# Autodesk Inventor assembly: REAR RIGHT BUKHEAD
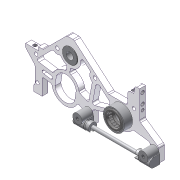
[picture p0: Inventor's stored thumbnail of the model, 180x180]
Saved by Autodesk Inventor 2016 (Build 200138000, 138)
## iProperties
Created: 2015-04-18
Part Number: REAR RIGHT BUKHEAD
Document SubType Name: Assembly
Designer: Station9
Author: Station9
## Documents named in this file (10)
- E:\worldskills Project\Project Archive\AD\AD-6(94.01.29)WSC2011\REAR RIGHT BUKHEAD.iam
- E:\worldskills Project\Project Archive\AD\AD-6(94.01.29)WSC2011\500-171.ipt
- E:\worldskills Project\Project Archive\AD\AD-6(94.01.29)WSC2011\500-172.ipt
- E:\worldskills Project\Project Archive\AD\AD-6(94.01.29)WSC2011\500-168.ipt
- E:\worldskills Project\Project Archive\AD\AD-6(94.01.29)WSC2011\500-160.ipt
- E:\worldskills Project\Project Archive\AD\AD-6(94.01.29)WSC2011\500-125.ipt
- E:\worldskills Project\Project Archive\AD\AD-6(94.01.29)WSC2011\500-169.ipt
- E:\worldskills Project\Project Archive\AD\AD-6(94.01.29)WSC2011\500-136.ipt
- E:\worldskills Project\Project Archive\AD\AD-6(94.01.29)WSC2011\Content Center\en-US\ISO 3245 (I)\ISO 3245 - 21 D - 12 x 16 x 7(1) I.ipt
- E:\worldskills Project\Project Archive\AD\AD-6(94.01.29)WSC2011\Bulkhead_RR.ipt
## Components (11 placed, 9 different names)
1. 500-171:1 — Mate:6, Mate:9, Mate:17, Mate:19
2. 500-172:1 — Mate:5, Mate:7, Mate:15, Mate:16, Mate:18
3. 500-168:1 — Mate:8, Mate:9, Mate:11, Angle:1
4. 500-160:1 — Mate:10, Mate:11, Angle:1
5. 500-125:1 — Insert:6
6. 500-169:1 — Mate:5, Mate:6, Mate:7, Mate:8, Mate:10, Mate:13, Mate:14
7. 500-136:1 — Insert:4, Insert:5
8. Bulkhead_RR:1 — Mate:16, Mate:17, Mate:18, Mate:19, Insert:5, Insert:6
9. 500-168:2 — Mate:13, Mate:15
10. 500-160:2 — Mate:14
11. ISO 3245 (I) 21 D - 12 x 16 x 7:1 — Insert:4
## Relationships (20: Mate 15, Insert 3, Angle 2)
- Mate:5: 500-172:1 ↔ 500-169:1
- Mate:6: 500-171:1 ↔ 500-169:1
- Mate:7: 500-172:1 ↔ 500-169:1
- Mate:8: 500-168:1 ↔ 500-169:1
- Mate:9: 500-171:1 ↔ 500-168:1
- Mate:10: 500-160:1 ↔ 500-169:1
- Mate:11: 500-168:1 ↔ 500-160:1
- Angle:1 (0 deg): 500-168:1 ↔ 500-160:1
- [Mate]: 500-168:2 ↔ 500-160:2
- [Angle] (0 deg): 500-168:2 ↔ 500-160:2
- Mate:13: 500-169:1 ↔ 500-168:2
- Mate:14: 500-169:1 ↔ 500-160:2
- Mate:15: 500-172:1 ↔ 500-168:2
- Insert:4: 500-136:1 ↔ ISO 3245 (I) 21 D - 12 x 16 x 7:1
- Mate:16: 500-172:1 ↔ Bulkhead_RR:1
- Mate:17: 500-171:1 ↔ Bulkhead_RR:1
- Mate:18: 500-172:1 ↔ Bulkhead_RR:1
- Mate:19: 500-171:1 ↔ Bulkhead_RR:1
- Insert:5: 500-136:1 ↔ Bulkhead_RR:1
- Insert:6: 500-125:1 ↔ Bulkhead_RR:1
## Named parameters: d20_d18 = 0 mm, d21_d19 = 0 deg
